# Autodesk Inventor assembly: SE. Chasis DC 2m
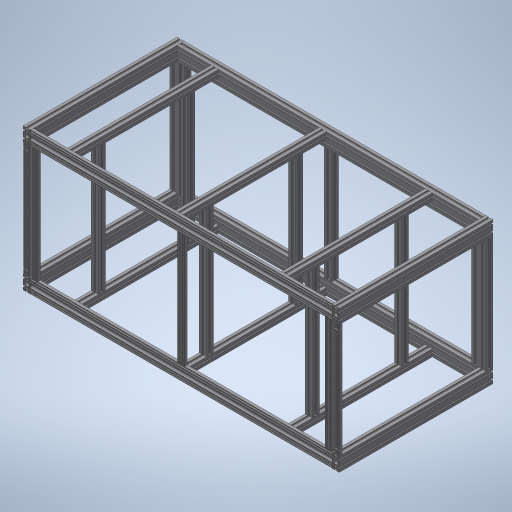
[picture p0: Inventor's stored thumbnail of the model, 512x512]
Saved by Autodesk Inventor 2024.2 (Build 282272000, 272)
## iProperties
Created: 2024-06-24
Part Number: SE. Chasis DC 2m
Material: Genérico
Document SubType Name: Assembly
Designer: jd.castellanosq
Author: jd.castellanosq
## Documents named in this file (9)
- I:\MICROMECANICA\ALTAS ENERGIAS\Deteccion de Muones\Detectores centelladores\Partes Detectores centelladores\Chasis DC\SE. Chasis DC 2m.iam
- I:\MICROMECANICA\ALTAS ENERGIAS\Deteccion de Muones\Detectores centelladores\Partes Detectores centelladores\Chasis DC\Partes Chasis DC\Perfil 45X90\Perfil 45X90-1501.ipt
- I:\MICROMECANICA\ALTAS ENERGIAS\Deteccion de Muones\Detectores centelladores\Partes Detectores centelladores\Chasis DC\Partes Chasis DC\Perfil 45X90.ipt
- I:\MICROMECANICA\ALTAS ENERGIAS\Deteccion de Muones\Detectores centelladores\Partes Detectores centelladores\Chasis DC\Partes Chasis DC\Perfil 45X90\Perfil 45X90-1000.ipt
- I:\MICROMECANICA\ALTAS ENERGIAS\Deteccion de Muones\Detectores centelladores\Partes Detectores centelladores\Chasis DC\Partes Chasis DC\Perfil 45X45\Perfil 45X45x910.ipt
- I:\MICROMECANICA\ALTAS ENERGIAS\Deteccion de Muones\Detectores centelladores\Partes Detectores centelladores\Chasis DC\Partes Chasis DC\Perfil 45X45.ipt
- I:\MICROMECANICA\ALTAS ENERGIAS\Deteccion de Muones\Detectores centelladores\Partes Detectores centelladores\Chasis DC\Partes Chasis DC\Perfil 45X45\Perfil 45X45X720.ipt
- I:\MICROMECANICA\ALTAS ENERGIAS\Deteccion de Muones\Detectores centelladores\Partes Detectores centelladores\Chasis DC\Partes Chasis DC\Perfil 45X45\Perfil 45X45-911.ipt
- I:\MICROMECANICA\ALTAS ENERGIAS\Deteccion de Muones\Detectores centelladores\Partes Detectores centelladores\Chasis DC\Partes Chasis DC\Perfil 45X90\Perfil 45X90-1502.ipt
## Components (26 placed, 6 different names)
1. Perfil 45X90-1502:13 — Mate:65, Flush:83, Flush:84, Flush:85, Flush:86, Mate:66, Flush:92, Mate:71, Flush:94, Mate:72, Flush:108, Mate:82, Mate:88, Flush:115
2. Perfil 45X90-1000:17 — Mate:65, Flush:83, Flush:84, Flush:95, Flush:99, Mate:74
3. Perfil 45X90-1000:18 — Flush:85, Flush:86, Mate:66, Mate:67, Flush:87, Flush:88, Flush:93, Flush:97
4. Perfil 45X90-1502:21 — Mate:67, Flush:87, Flush:88, Flush:96, Mate:73, Flush:98, Flush:109, Flush:110, Mate:85, Mate:87, Flush:114
5. Perfil 45X45x910:39 — Flush:109
6. Perfil 45X45x910:40 — Flush:110, Mate:82
7. Perfil 45X45x910:41 — Flush:108
8. Perfil 45X45X720:45
9. Perfil 45X45X720:46
10. Perfil 45X45X720:47 — Mate:86
11. Perfil 45X45X720:48 — Mate:85, Mate:86
12. Perfil 45X45X720:49
13. Perfil 45X45X720:50
14. Perfil 45X90-1502:14 — Flush:106, Flush:107, Mate:78
15. Perfil 45X90-1000:19 — Flush:100, Flush:101, Mate:75, Mate:76, Flush:107, Mate:78
16. Perfil 45X90-1000:20 — Flush:103, Flush:104, Flush:105
17. Perfil 45X90-1502:28 — Mate:76, Flush:102, Mate:77, Flush:105, Flush:112, Mate:89, Mate:90
18. Perfil 45X90-1501:9 — Flush:96, Flush:97, Mate:73, Flush:103, Flush:104
19. Perfil 45X90-1501:10 — Flush:92, Mate:71, Flush:93
20. Perfil 45X90-1501:11 — Flush:94, Mate:72, Flush:95, Flush:106
21. Perfil 45X90-1501:12 — Flush:98, Flush:99, Mate:74, Flush:100, Flush:101, Mate:75, Flush:102, Mate:77
22. Perfil 45X45x910:42 — Mate:89
23. Perfil 45X45x910:43 — Flush:112
24. Perfil 45X45x910:44 — Mate:90
25. Perfil 45X45-911:51 — Mate:87, Flush:114
26. Perfil 45X45-911:52 — Mate:88, Flush:115
## Relationships (74: Flush 45, Mate 29)
- [Mate]: Perfil 45X90-1502:13
- [Mate]: Perfil 45X90-1502:13
- [Flush]: Perfil 45X90-1502:13
- [Flush]: Perfil 45X45X720:47 ↔ Perfil 45X45X720:48
- [Flush]: Perfil 45X45X720:47 ↔ Perfil 45X45X720:48
- [Flush]: Perfil 45X45X720:45 ↔ Perfil 45X45X720:46
- [Flush]: Perfil 45X45X720:45 ↔ Perfil 45X45X720:46
- [Flush]: Perfil 45X45x910:41 ↔ Perfil 45X45X720:48
- [Flush]: Perfil 45X45X720:45 ↔ Perfil 45X45X720:48
- [Flush]: Perfil 45X45X720:46 ↔ Perfil 45X45X720:47
- [Flush]: Perfil 45X45x910:39 ↔ Perfil 45X45X720:50
- [Flush]: Perfil 45X45X720:48 ↔ Perfil 45X45X720:50
- [Flush]: Perfil 45X45x910:39 ↔ Perfil 45X45X720:49
- [Flush]: Perfil 45X45X720:47 ↔ Perfil 45X45X720:49
- [Mate]: Perfil 45X45X720:50 ↔ Perfil 45X45x910:42
- [Flush]: Perfil 45X45X720:50 ↔ Perfil 45X45x910:42
- [Mate]: Perfil 45X90-1502:28 ↔ Perfil 45X45x910:43
- [Flush]: Perfil 45X45X720:45 ↔ Perfil 45X45x910:43
- [Mate]: Perfil 45X45X720:48 ↔ Perfil 45X45x910:44
- [Flush]: Perfil 45X45X720:48 ↔ Perfil 45X45x910:44
- Mate:65: Perfil 45X90-1502:13 ↔ Perfil 45X90-1000:17
- Flush:83: Perfil 45X90-1502:13 ↔ Perfil 45X90-1000:17
- Flush:84: Perfil 45X90-1502:13 ↔ Perfil 45X90-1000:17
- Flush:85: Perfil 45X90-1502:13 ↔ Perfil 45X90-1000:18
- Flush:86: Perfil 45X90-1502:13 ↔ Perfil 45X90-1000:18
- Mate:66: Perfil 45X90-1502:13 ↔ Perfil 45X90-1000:18
- Mate:67: Perfil 45X90-1000:18 ↔ Perfil 45X90-1502:21
- Flush:87: Perfil 45X90-1000:18 ↔ Perfil 45X90-1502:21
- Flush:88: Perfil 45X90-1000:18 ↔ Perfil 45X90-1502:21
- [Mate]: Perfil 45X90-1502:13 ↔ Perfil 45X45x910:39
- [Mate]: Perfil 45X90-1502:13 ↔ Perfil 45X45x910:41
- Flush:92: Perfil 45X90-1502:13 ↔ Perfil 45X90-1501:10
- Mate:71: Perfil 45X90-1502:13 ↔ Perfil 45X90-1501:10
- Flush:93: Perfil 45X90-1000:18 ↔ Perfil 45X90-1501:10
- Flush:94: Perfil 45X90-1502:13 ↔ Perfil 45X90-1501:11
- Mate:72: Perfil 45X90-1502:13 ↔ Perfil 45X90-1501:11
- Flush:95: Perfil 45X90-1000:17 ↔ Perfil 45X90-1501:11
- Flush:96: Perfil 45X90-1502:21 ↔ Perfil 45X90-1501:9
- Flush:97: Perfil 45X90-1000:18 ↔ Perfil 45X90-1501:9
- Mate:73: Perfil 45X90-1502:21 ↔ Perfil 45X90-1501:9
- Flush:98: Perfil 45X90-1502:21 ↔ Perfil 45X90-1501:12
- Flush:99: Perfil 45X90-1000:17 ↔ Perfil 45X90-1501:12
- Mate:74: Perfil 45X90-1000:17 ↔ Perfil 45X90-1501:12
- Flush:100: Perfil 45X90-1000:19 ↔ Perfil 45X90-1501:12
- Flush:101: Perfil 45X90-1000:19 ↔ Perfil 45X90-1501:12
- Mate:75: Perfil 45X90-1000:19 ↔ Perfil 45X90-1501:12
- Mate:76: Perfil 45X90-1000:19 ↔ Perfil 45X90-1502:28
- Flush:102: Perfil 45X90-1502:28 ↔ Perfil 45X90-1501:12
- Mate:77: Perfil 45X90-1502:28 ↔ Perfil 45X90-1501:12
- Flush:103: Perfil 45X90-1000:20 ↔ Perfil 45X90-1501:9
- Flush:104: Perfil 45X90-1000:20 ↔ Perfil 45X90-1501:9
- Flush:105: Perfil 45X90-1000:20 ↔ Perfil 45X90-1502:28
- Flush:106: Perfil 45X90-1502:14 ↔ Perfil 45X90-1501:11
- Flush:107: Perfil 45X90-1502:14 ↔ Perfil 45X90-1000:19
- Mate:78: Perfil 45X90-1502:14 ↔ Perfil 45X90-1000:19
- Flush:108: Perfil 45X90-1502:13 ↔ Perfil 45X45x910:41
- [Mate]: Perfil 45X45x910:41 ↔ Perfil 45X45X720:47
- Flush:109: Perfil 45X90-1502:21 ↔ Perfil 45X45x910:39
- [Mate]: Perfil 45X45x910:39 ↔ Perfil 45X45X720:50
- [Mate]: Perfil 45X45x910:39 ↔ Perfil 45X45X720:49
- Flush:110: Perfil 45X90-1502:21 ↔ Perfil 45X45x910:40
- Mate:82: Perfil 45X90-1502:13 ↔ Perfil 45X45x910:40
- [Mate]: Perfil 45X45x910:40 ↔ Perfil 45X45X720:46
- [Flush]: Perfil 45X45x910:40 ↔ Perfil 45X45X720:46
- Flush:112: Perfil 45X90-1502:28 ↔ Perfil 45X45x910:43
- [Flush]: Perfil 45X45X720:45 ↔ Perfil 45X45x910:43
- Mate:85 (150 mm): Perfil 45X90-1502:21 ↔ Perfil 45X45X720:48
- Mate:86 (-610 mm): Perfil 45X45X720:47 ↔ Perfil 45X45X720:48
- Mate:87: Perfil 45X90-1502:21 ↔ Perfil 45X45-911:51
- Flush:114: Perfil 45X90-1502:21 ↔ Perfil 45X45-911:51
- Mate:88: Perfil 45X90-1502:13 ↔ Perfil 45X45-911:52
- Flush:115: Perfil 45X90-1502:13 ↔ Perfil 45X45-911:52
- Mate:89: Perfil 45X90-1502:28 ↔ Perfil 45X45x910:42
- Mate:90: Perfil 45X90-1502:28 ↔ Perfil 45X45x910:44
